# Autodesk Inventor assembly: growbox
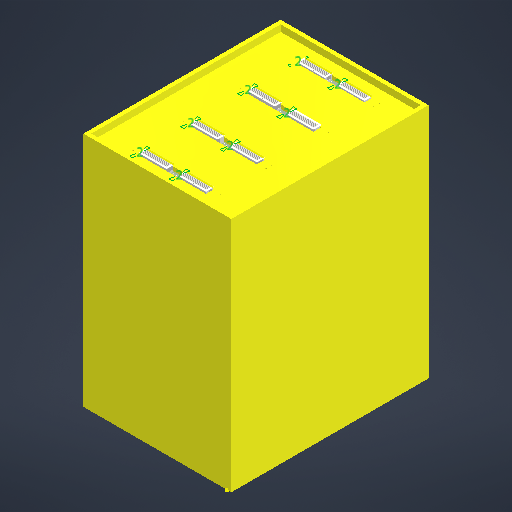
[picture p0: Inventor's stored thumbnail of the model, 512x512]
Saved by Autodesk Inventor 2027.1 (Build 311270010, 270A)
## iProperties
Created: 2026-10-02
Part Number: growbox
Document SubType Name: Assembly
Designer: Arik
Author: Arik
## Documents named in this file (4)
- C:\Users\Arik\Desktop\microgrowery\docs\CAD\growbox.iam
- C:\Users\Arik\Desktop\microgrowery\docs\CAD\box.ipt
- C:\Users\Arik\Desktop\microgrowery\docs\CAD\led_board\led_board.ipt
- C:\Users\Arik\Desktop\microgrowery\docs\CAD\heatsink.ipt
## Components (13 placed, 3 different names)
1. box:1 — Mate:1, Mate:2, Mate:3, Mate:4, Mate:5, Mate:6, Mate:7, Mate:8, Mate:9, Mate:10, Mate:11, Mate:12, Mate:14, Mate:15, Mate:16, Mate:18, Mate:20, Mate:21, Mate:23, Mate:24, Mate:26, Mate:27, Mate:29, Mate:30, Mate:32, Mate:33, Mate:35, Mate:36
2. led_board:1 — Mate:1, Mate:2, Mate:12, Mate:13, Mate:17
3. led_board:2 — Mate:3, Mate:4, Mate:11, Mate:19, Mate:22
4. led_board:3 — Mate:5, Mate:6, Mate:10, Mate:25, Mate:28
5. led_board:4 — Mate:7, Mate:8, Mate:9, Mate:31, Mate:34
6. heatsink:1 — Mate:13, Mate:14, Mate:15
7. heatsink:2 — Mate:16, Mate:17, Mate:18
8. heatsink:3 — Mate:19, Mate:20, Mate:21
9. heatsink:4 — Mate:22, Mate:23, Mate:24
10. heatsink:5 — Mate:25, Mate:26, Mate:27
11. heatsink:6 — Mate:28, Mate:29, Mate:30
12. heatsink:7 — Mate:31, Mate:32, Mate:33
13. heatsink:8 — Mate:34, Mate:35, Mate:36
## Relationships (36: Mate 36)
- Mate:1: box:1 ↔ led_board:1
- Mate:2: box:1 ↔ led_board:1
- Mate:3: box:1 ↔ led_board:2
- Mate:4: box:1 ↔ led_board:2
- Mate:5: box:1 ↔ led_board:3
- Mate:6: box:1 ↔ led_board:3
- Mate:7: box:1 ↔ led_board:4
- Mate:8: box:1 ↔ led_board:4
- Mate:9: box:1 ↔ led_board:4
- Mate:10: box:1 ↔ led_board:3
- Mate:11: box:1 ↔ led_board:2
- Mate:12: box:1 ↔ led_board:1
- Mate:13: led_board:1 ↔ heatsink:1
- Mate:14: box:1 ↔ heatsink:1
- Mate:15: box:1 ↔ heatsink:1
- Mate:16: box:1 ↔ heatsink:2
- Mate:17: led_board:1 ↔ heatsink:2
- Mate:18: box:1 ↔ heatsink:2
- Mate:19: led_board:2 ↔ heatsink:3
- Mate:20: box:1 ↔ heatsink:3
- Mate:21: box:1 ↔ heatsink:3
- Mate:22: led_board:2 ↔ heatsink:4
- Mate:23: box:1 ↔ heatsink:4
- Mate:24: box:1 ↔ heatsink:4
- Mate:25: led_board:3 ↔ heatsink:5
- Mate:26: box:1 ↔ heatsink:5
- Mate:27: box:1 ↔ heatsink:5
- Mate:28: led_board:3 ↔ heatsink:6
- Mate:29: box:1 ↔ heatsink:6
- Mate:30: box:1 ↔ heatsink:6
- Mate:31: led_board:4 ↔ heatsink:7
- Mate:32: box:1 ↔ heatsink:7
- Mate:33: box:1 ↔ heatsink:7
- Mate:34: led_board:4 ↔ heatsink:8
- Mate:35: box:1 ↔ heatsink:8
- Mate:36: box:1 ↔ heatsink:8
